# Autodesk Inventor assembly: drivebay
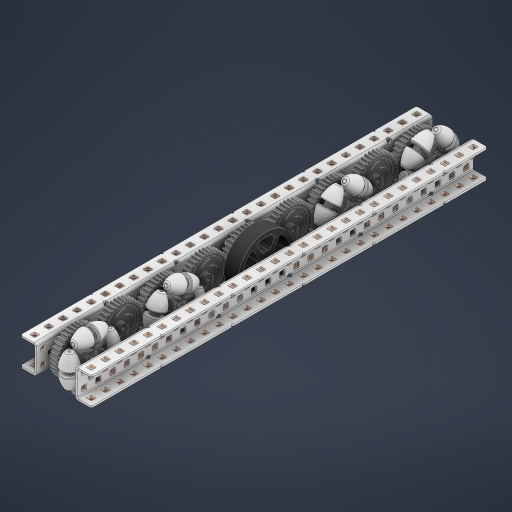
[picture p0: Inventor's stored thumbnail of the model, 512x512]
Saved by Autodesk Inventor 2024 (Build 280153000, 153)
## iProperties
Created: 2024-01-13
Part Number: drivebay
Document SubType Name: Assembly
Designer: avere
Author: avere
## Documents named in this file (6)
- C:\Users\avere\Documents\rbp_cad\zoomba_v0.3\drivebay.iam
- C:\Users\avere\Documents\rbp_cad\VEX-CAD-Inventor-1.41\Structure\C Channel\Aluminum 1x2x1\Alu C 1x2x1x28.ipt
- C:\Users\avere\Documents\rbp_cad\zoomba_v0.3\wheel_hub.iam
- C:\Users\avere\Documents\rbp_cad\VEX-CAD-Inventor-1.41\Structure\C Channel\Aluminum 1x2x1\Alu C 1x2x1x5.ipt
- C:\Users\avere\Documents\rbp_cad\zoomba_v0.3\flex_wheel_hub.iam
- C:\Users\avere\Documents\rbp_cad\VEX-CAD-Inventor-1.41\Motion\Gears\LS 36T Gear.ipt
## Components (12 placed, 5 different names)
1. Alu C 1x2x1x28:1 — Insert:1, Mate:1, Insert:12, Insert:13, Insert:14, Insert:15, Insert:16, Insert:17, Insert:18, Insert:19, Insert:20
2. wheel_hub:1 [sub-assembly] — Insert:12
3. Alu C 1x2x1x28:2
4. Alu C 1x2x1x5:1 — Insert:1, Mate:1
5. wheel_hub:2 [sub-assembly] — Insert:13
6. wheel_hub:4 [sub-assembly] — Insert:15
7. wheel_hub:5 [sub-assembly] — Insert:16
8. flex_wheel_hub:1 [sub-assembly] — Insert:14
9. LS 36T Gear:1 — Insert:17
10. LS 36T Gear:2 — Insert:18
11. LS 36T Gear:3 — Insert:19
12. LS 36T Gear:4 — Insert:20
## Relationships (11: Insert 10, Mate 1)
- Insert:1: Alu C 1x2x1x28:1 ↔ Alu C 1x2x1x5:1
- Mate:1: Alu C 1x2x1x28:1 ↔ Alu C 1x2x1x5:1
- Insert:12 (4.7625 mm): Alu C 1x2x1x28:1 ↔ wheel_hub:1
- Insert:13 (4.7625 mm): Alu C 1x2x1x28:1 ↔ wheel_hub:2
- Insert:14 (4.7625 mm): Alu C 1x2x1x28:1 ↔ flex_wheel_hub:1
- Insert:15 (4.7625 mm): Alu C 1x2x1x28:1 ↔ wheel_hub:4
- Insert:16 (4.7625 mm): Alu C 1x2x1x28:1 ↔ wheel_hub:5
- Insert:17 (4.7625 mm): Alu C 1x2x1x28:1 ↔ LS 36T Gear:1
- Insert:18 (4.7625 mm): Alu C 1x2x1x28:1 ↔ LS 36T Gear:2
- Insert:19 (4.7625 mm): Alu C 1x2x1x28:1 ↔ LS 36T Gear:3
- Insert:20 (4.7625 mm): Alu C 1x2x1x28:1 ↔ LS 36T Gear:4
